# Autodesk Inventor assembly: Bearings
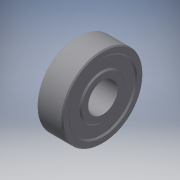
[picture p0: Inventor's stored thumbnail of the model, 180x180]
Saved by Autodesk Inventor 2019 (Build 230136000, 136)
## iProperties
Created: 2020-12-03
Part Number: Bearings
Document SubType Name: Assembly
Designer: Anass Hamdi
Author: Anass Hamdi
## Documents named in this file (7)
- C:\Users\Anass Hamdi\OneDrive - Vrije Universiteit Brussel\Documenten\Inventor\Anass Hamdi Project\Bearings.iam
- C:\Users\Anass Hamdi\OneDrive - Vrije Universiteit Brussel\Documenten\Inventor\Anass Hamdi Project\Bearings_Retainer.ipt
- C:\Users\Anass Hamdi\OneDrive - Vrije Universiteit Brussel\Documenten\Inventor\Anass Hamdi Project\Bearings _Ball.ipt
- C:\Users\Anass Hamdi\OneDrive - Vrije Universiteit Brussel\Documenten\Inventor\Anass Hamdi Project\Bearings_InnerRace.ipt
- C:\Users\Anass Hamdi\OneDrive - Vrije Universiteit Brussel\Documenten\Inventor\Anass Hamdi Project\Bearings_OuterRace.ipt
- C:\Users\Anass Hamdi\OneDrive - Vrije Universiteit Brussel\Documenten\Inventor\Anass Hamdi Project\Bearings_Shields.ipt
- C:\Users\Anass Hamdi\OneDrive - Vrije Universiteit Brussel\Documenten\Inventor\Anass Hamdi Project\Bearings - Shields.ipt
## Components (11 placed, 6 different names)
1. Bearings _Ball:1 — Ball:4
2. Bearings_InnerRace:1 — Rotational:2
3. Bearings_OuterRace:1 — Rotational:2, Rotational:3, Rigid:1, Rigid:2
4. Bearings_Retainer:1 — Rotational:3, Ball:1, Ball:2, Ball:3, Ball:4, Ball:5, Ball:6
5. Bearings_Shields:1 — Rigid:2
6. Bearings _Ball:2 — Ball:3
7. Bearings _Ball:3 — Ball:2
8. Bearings _Ball:4 — Ball:1
9. Bearings _Ball:5 — Ball:5
10. Bearings _Ball:6 — Ball:6
11. Bearings - Shields:1 — Rigid:1
## Relationships (10: BallJoint 6, RevoluteJoint 2, WeldJoint 2)
- Rotational:2 [RevoluteJoint]: Bearings_InnerRace:1 ↔ Bearings_OuterRace:1
- Rotational:3 [RevoluteJoint]: Bearings_OuterRace:1 ↔ Bearings_Retainer:1
- Ball:1: Bearings_Retainer:1 ↔ Bearings _Ball:4
- Ball:2: Bearings_Retainer:1 ↔ Bearings _Ball:3
- Ball:3: Bearings_Retainer:1 ↔ Bearings _Ball:2
- Ball:4: Bearings _Ball:1 ↔ Bearings_Retainer:1
- Ball:5: Bearings_Retainer:1 ↔ Bearings _Ball:5
- Ball:6: Bearings_Retainer:1 ↔ Bearings _Ball:6
- Rigid:1 [WeldJoint]: Bearings_OuterRace:1 ↔ Bearings - Shields:1
- Rigid:2 [WeldJoint]: Bearings_OuterRace:1 ↔ Bearings_Shields:1
